# Autodesk Inventor assembly: ENSAMBLE GENERAL M 2021-4.5L
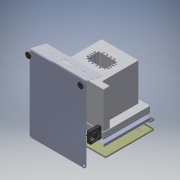
[picture p0: Inventor's stored thumbnail of the model, 180x180]
Saved by Autodesk Inventor 2017 (Build 210142000, 142)
## iProperties
Created: 2021-03-24
Part Number: ENSAMBLE GENERAL M 2021-4.5L
Description: STEP AP214
Document SubType Name: Assembly
Designer: USUARIO
Sending System: SolidWorks 2013
Preprocessor: SwSTEP 2.0
Title: ENSAMBLE GENERAL M 2021-4.5L.STEP
Revision Number: ANY
## Documents named in this file (18)
- D:\Laboratorio\Mufla\2021\Mufla 4.5L Psoc MYC Lab #0045885XX OP202145\Modelo\ENSAMBLE GENERAL M 2021-4.5L.iam
- D:\Laboratorio\Mufla\2021\Mufla 4.5L Psoc MYC Lab #0045885XX OP202145\Modelo\ENSAMBLE CUERPO M 2021-4.5L.iam
- D:\Laboratorio\Mufla\2021\Mufla 4.5L Psoc MYC Lab #0045885XX OP202145\Modelo\ENSAMBLE PUERTA M 2021-4.5L.iam
- D:\Laboratorio\Mufla\2021\Mufla 4.5L Psoc MYC Lab #0045885XX OP202145\Modelo\TAPA FRONTAL M 2021-4.5L.ipt
- D:\Laboratorio\Mufla\2021\Mufla 4.5L Psoc MYC Lab #0045885XX OP202145\Modelo\TAPA BASE M 2021-4.5L.ipt
- D:\Laboratorio\Mufla\2021\Mufla 4.5L Psoc MYC Lab #0045885XX OP202145\Modelo\VENTILADOR 9X9.ipt
- D:\Laboratorio\Mufla\2021\Mufla 4.5L Psoc MYC Lab #0045885XX OP202145\Modelo\TAPA INFERIOR M 2021-4.5L.ipt
- D:\Laboratorio\Mufla\2021\Mufla 4.5L Psoc MYC Lab #0045885XX OP202145\Modelo\COMPLEMENTO BASE M 2021-4.5L.ipt
- D:\Laboratorio\Mufla\2021\Mufla 4.5L Psoc MYC Lab #0045885XX OP202145\Modelo\PG-13,5.ipt
- D:\Laboratorio\Mufla\2021\Mufla 4.5L Psoc MYC Lab #0045885XX OP202145\Modelo\BRAKER.ipt
- D:\Laboratorio\Mufla\2021\Mufla 4.5L Psoc MYC Lab #0045885XX OP202145\Modelo\SUJECION BREAKER M 2021-4.5L.ipt
- D:\Laboratorio\Mufla\2021\Mufla 4.5L Psoc MYC Lab #0045885XX OP202145\Modelo\TAPA POSTERIOR-INTERIOR M 2021-4.5L.ipt
- D:\Laboratorio\Mufla\2021\Mufla 4.5L Psoc MYC Lab #0045885XX OP202145\Modelo\TAPA POSTERIOR M 2021-4.5L.ipt
- D:\Laboratorio\Mufla\2021\Mufla 4.5L Psoc MYC Lab #0045885XX OP202145\Modelo\PATA 5-16.ipt
- D:\Laboratorio\Mufla\2021\Mufla 4.5L Psoc MYC Lab #0045885XX OP202145\Modelo\TUERCA REMACHABLE 0,3125.ipt
- D:\Laboratorio\Mufla\2021\Mufla 4.5L Psoc MYC Lab #0045885XX OP202145\Modelo\COMPLEMENTO CUERPO INTERIOR M 2020- 4L (B).ipt
- D:\Laboratorio\Mufla\2021\Mufla 4.5L Psoc MYC Lab #0045885XX OP202145\Modelo\EnsambleAislante.iam
- D:\Laboratorio\Mufla\2021\Mufla 4.5L Psoc MYC Lab #0045885XX OP202145\Modelo\Resistencia2.ipt
## Components (25 placed, 22 different names)
1. ENSAMBLE CUERPO M 2021-4.5L_1 [sub-assembly] — Mate:3, Flush:1
2. ENSAMBLE PUERTA M 2021-4.5L_2 [sub-assembly] — Flush:3, Mate:4
3. TAPA FRONTAL M 2021-4.5L_3 — Flush:3, Mate:4
4. TAPA BASE M 2021-4.5L_4
5. VENTILADOR 9X9_5
6. VENTILADOR 9X9_6
7. TAPA INFERIOR M 2021-4.5L_7
8. COMPLEMENTO BASE M 2021-4.5L_8
9. PG-13,5_9
10. BRAKER_10
11. SUJECION BREAKER M 2021-4.5L_11
12. TAPA POSTERIOR-INTERIOR M 2021-4.5L_12
13. TAPA POSTERIOR M 2021-4.5L_13
14. PATA 5-16_14
15. PATA 5-16_15
16. TUERCA REMACHABLE 0,3125_16
17. TUERCA REMACHABLE 0,3125_17
18. TUERCA REMACHABLE 0,3125_18
19. BRAKER_19
20. COMPLEMENTO CUERPO INTERIOR M 2020- 4L (B)_20
21. EnsambleAislante:1 [sub-assembly] — Mate:3, Flush:1, Insert:1, Insert:2, Insert:3, Insert:4
22. Resistencia2:1 — Insert:2
23. Resistencia2:2 — Insert:1
24. Resistencia2:3 — Insert:4
25. Resistencia2:4 — Insert:3
## Relationships (8: Insert 4, Mate 2, Flush 2)
- Mate:3: ENSAMBLE CUERPO M 2021-4.5L_1 ↔ EnsambleAislante:1
- Flush:1: ENSAMBLE CUERPO M 2021-4.5L_1 ↔ EnsambleAislante:1
- Flush:3: ENSAMBLE PUERTA M 2021-4.5L_2 ↔ TAPA FRONTAL M 2021-4.5L_3
- Mate:4 (5 mm): ENSAMBLE PUERTA M 2021-4.5L_2 ↔ TAPA FRONTAL M 2021-4.5L_3
- Insert:1: EnsambleAislante:1 ↔ Resistencia2:2
- Insert:2: EnsambleAislante:1 ↔ Resistencia2:1
- Insert:3: EnsambleAislante:1 ↔ Resistencia2:4
- Insert:4: EnsambleAislante:1 ↔ Resistencia2:3
